# Autodesk Inventor assembly: BASE
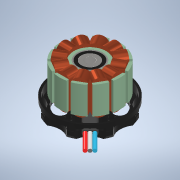
[picture p0: Inventor's stored thumbnail of the model, 180x180]
Saved by Autodesk Inventor 2022 (Build 260153000, 153)
## iProperties
Created: 2022-07-25
Part Number: BASE
Document SubType Name: Assembly
Designer: Nathan Cai
Author: Nathan Cai
## Documents named in this file (7)
- C:\Users\Nathan Cai\Documents\Inventor\Asorted Parts\Aerosky MC4230 630KV\BASE.iam
- C:\Users\Nathan Cai\Documents\Inventor\Asorted Parts\Aerosky MC4230 630KV\BASE.ipt
- C:\Users\Nathan Cai\Documents\Inventor\Asorted Parts\Aerosky MC4230 630KV\BEARING.ipt
- C:\Users\Nathan Cai\Documents\Inventor\Asorted Parts\Aerosky MC4230 630KV\SLEEVE.ipt
- C:\Users\Nathan Cai\Documents\Inventor\Asorted Parts\Aerosky MC4230 630KV\STATOR.ipt
- C:\Users\Nathan Cai\Documents\Inventor\Asorted Parts\Aerosky MC4230 630KV\COILS.ipt
- C:\Users\Nathan Cai\Documents\Inventor\Asorted Parts\Aerosky MC4230 630KV\CABLE.ipt
## Components (18 placed, 6 different names)
1. BASE:1 — Mate:1, Mate:2, Mate:3, Mate:4, Mate:5, Mate:6, Flush:1, Mate:10, Mate:11, Mate:12
2. BEARING:1 — Mate:3, Mate:4
3. BEARING:2 — Mate:1, Mate:2
4. SLEEVE:1 — Mate:5, Mate:6, Mate:7
5. STATOR:1 — Mate:7, Flush:1, Mate:8, Tangent:1, Mate:9
6. CABLE:1 — Mate:10, Flush:2
7. COILS:1 — Mate:8, Tangent:1, Mate:9
8. COILS:2
9. COILS:3
10. COILS:4
11. COILS:5
12. COILS:6
13. COILS:7
14. COILS:8
15. COILS:9
16. COILS:10
17. COILS:11
18. COILS:12
## Component patterns: (12 elements, first: COILS:1)
## Relationships (15: Mate 12, Flush 2, Tangent 1)
- Mate:1: BASE:1 ↔ BEARING:2
- Mate:2: BASE:1 ↔ BEARING:2
- Mate:3: BASE:1 ↔ BEARING:1
- Mate:4: BASE:1 ↔ BEARING:1
- Mate:5: BASE:1 ↔ SLEEVE:1
- Mate:6: BASE:1 ↔ SLEEVE:1
- Mate:7: SLEEVE:1 ↔ STATOR:1
- Flush:1: BASE:1 ↔ STATOR:1
- Mate:8: STATOR:1 ↔ COILS:1
- Tangent:1: STATOR:1 ↔ COILS:1
- Mate:9 (3 mm): STATOR:1 ↔ COILS:1
- Mate:10: BASE:1 ↔ CABLE:1
- Mate:11: BASE:1
- Mate:12: BASE:1
- Flush:2: CABLE:1
